# Autodesk Inventor assembly: Lower skin assembly
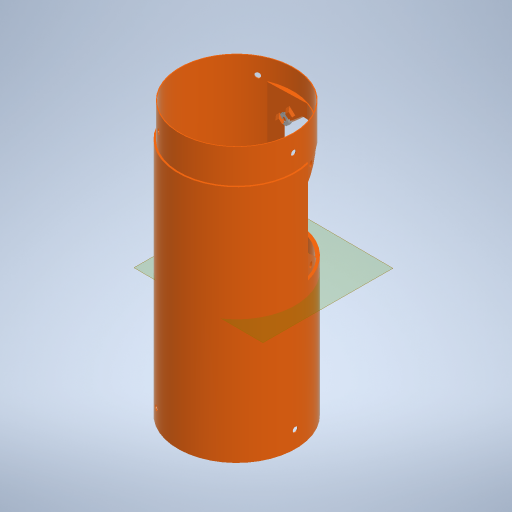
[picture p0: Inventor's stored thumbnail of the model, 512x512]
Saved by Autodesk Inventor 2024 (Build 280153000, 153)
## iProperties
Created: 2024-04-27
Part Number: Lower skin assembly
Document SubType Name: Assembly
Designer: auror
Author: auror
## Documents named in this file (4)
- C:\Users\auror\Documents\TU Delft\DARE\Git\Scrambler-2-CAD\Autodesk\Lower skin assembly.iam
- C:\Users\auror\Documents\TU Delft\DARE\Git\Scrambler-2-CAD\Autodesk\Electronics Door.ipt
- C:\Users\auror\Documents\TU Delft\DARE\Git\Scrambler-2-CAD\Autodesk\Lower skin.ipt
- C:\Users\auror\Documents\TU Delft\DARE\Git\Scrambler-2-CAD\Autodesk\Nut.ipt
## Components (6 placed, 3 different names)
1. Electronics Door:1 — Mate:24
2. Lower skin:1 — Mate:13, Mate:14, Mate:15, Mate:16, Mate:17, Mate:18, Mate:19, Mate:20, Mate:21, Mate:22, Mate:23, Mate:24
3. AS 1112 (2) - Metric M3  Type 5:1 — Mate:13, Mate:14, Mate:15
4. AS 1112 (2) - Metric M3  Type 5:2 — Mate:16, Mate:17, Mate:18
5. AS 1112 (2) - Metric M3  Type 5:3 — Mate:19, Mate:20, Mate:21
6. AS 1112 (2) - Metric M3  Type 5:4 — Mate:22, Mate:23
## Relationships (12: Mate 12)
- Mate:13: Lower skin:1 ↔ AS 1112 (2) - Metric M3  Type 5:1
- Mate:14: Lower skin:1 ↔ AS 1112 (2) - Metric M3  Type 5:1
- Mate:15: Lower skin:1 ↔ AS 1112 (2) - Metric M3  Type 5:1
- Mate:16: Lower skin:1 ↔ AS 1112 (2) - Metric M3  Type 5:2
- Mate:17: Lower skin:1 ↔ AS 1112 (2) - Metric M3  Type 5:2
- Mate:18: Lower skin:1 ↔ AS 1112 (2) - Metric M3  Type 5:2
- Mate:19: Lower skin:1 ↔ AS 1112 (2) - Metric M3  Type 5:3
- Mate:20: Lower skin:1 ↔ AS 1112 (2) - Metric M3  Type 5:3
- Mate:21: Lower skin:1 ↔ AS 1112 (2) - Metric M3  Type 5:3
- Mate:22: Lower skin:1 ↔ AS 1112 (2) - Metric M3  Type 5:4
- Mate:23: Lower skin:1 ↔ AS 1112 (2) - Metric M3  Type 5:4
- Mate:24: Electronics Door:1 ↔ Lower skin:1
